# Autodesk Inventor assembly: MACHINEVISE
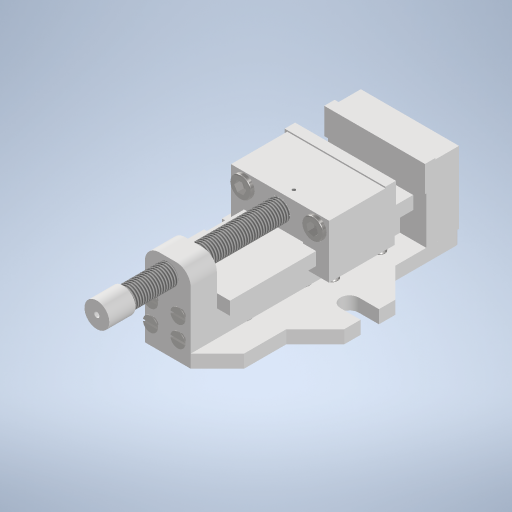
[picture p0: Inventor's stored thumbnail of the model, 512x512]
Saved by Autodesk Inventor 2024 (Build 280153000, 153)
## iProperties
Created: 2023-05-10
Part Number: MACHINEVISE
Document SubType Name: Assembly
Designer: Raj
Author: Raj
## Documents named in this file (16)
- D:\New folder\assembly 2\Assembly\MACHINEVISE.iam
- D:\New folder\assembly 2\Groundplate (1).ipt
- D:\New folder\assembly 2\Spindlesocket.ipt
- D:\New folder\assembly 2\Feste Backe (2).ipt
- D:\New folder\assembly 2\Fuhrung.ipt
- D:\New folder\assembly 2\Lose Backe.ipt
- D:\New folder\assembly 2\Spannbacke(n).ipt
- D:\New folder\assembly 2\Trapezspindle.ipt
- D:\New folder\assembly 2\Druckhulse.ipt
- D:\New folder\assembly 2\Fuhrungschiene(n).ipt
- C:\Users\USER\OneDrive\Documents\Inventor\Content Center Files\R2024\en-US\DIN 963\DIN 963 - M8 x 25.ipt
- C:\Users\USER\OneDrive\Documents\Inventor\Content Center Files\R2024\en-US\DIN 963\DIN 963 - M6 x 25.ipt
- C:\Users\USER\OneDrive\Documents\Inventor\Content Center Files\R2024\en-US\DIN 963\DIN 963 - M6 x 40.ipt
- C:\Users\USER\OneDrive\Documents\Inventor\Content Center Files\R2024\en-US\DIN 963\DIN 963 - M6 x 20.ipt
- C:\Users\USER\OneDrive\Documents\Inventor\Content Center Files\R2024\en-US\DIN 963\DIN 963 - M5 x 16.ipt
- C:\Users\USER\OneDrive\Documents\Inventor\Content Center Files\R2024\en-US\DIN 912\DIN 912 - M10 x 1.5 x 45 x 32.ipt
## Components (32 placed, 15 different names)
1. Groundplate (1):1 — Mate:1, Flush:1, Mate:2, Mate:3, Mate:4, Flush:2, Mate:7, Insert:13, Insert:14, Insert:15, Insert:16, Insert:17, Insert:18
2. Spindlesocket:1 — Mate:1, Flush:1, Mate:2, Mate:5, Mate:10, Insert:7, Insert:8, Insert:9, Insert:10
3. Fuhrung:1 — Mate:3, Mate:4, Mate:5, Mate:6, Mate:9
4. Feste Backe (2):1 — Mate:6, Flush:2, Mate:7, Mate:11, Mate:12, Mate:13, Insert:2, Insert:3, Insert:4, Insert:5, Insert:6
5. Lose Backe:1 — Mate:9, Mate:10, Insert:1, Mate:14, Mate:15, Mate:16, Mate:17, Mate:18, Mate:19, Mate:20, Mate:21, Mate:22, Mate:23, Mate:24, Insert:11, Insert:12
6. Trapezspindle:1 — Insert:1
7. Spannbacke(n):1 — Mate:11, Mate:12, Mate:13
8. Spannbacke(n):2 — Mate:14, Mate:15, Mate:16
9. Druckhulse:1 — Mate:17, Mate:18
10. Fuhrungschiene(n):1 — Mate:19, Mate:20, Mate:21, Insert:19, Insert:20
11. Fuhrungschiene(n):2 — Mate:22, Mate:23, Mate:24, Insert:21, Insert:22
12. DIN 963 - replaced by DIN EN ISO 2009 M8 x 25:1 — Insert:2
13. DIN 963 - replaced by DIN EN ISO 2009 M8 x 25:2 — Insert:3
14. DIN 963 - replaced by DIN EN ISO 2009 M8 x 25:3 — Insert:4
15. DIN 963 - replaced by DIN EN ISO 2009 M6 x 25:1 — Insert:5
16. DIN 963 - replaced by DIN EN ISO 2009 M6 x 25:2 — Insert:6
17. DIN 963 - replaced by DIN EN ISO 2009 M6 x 40:1 — Insert:7
18. DIN 963 - replaced by DIN EN ISO 2009 M6 x 40:2 — Insert:8
19. DIN 963 - replaced by DIN EN ISO 2009 M6 x 40:3 — Insert:10
20. DIN 963 - replaced by DIN EN ISO 2009 M6 x 40:4 — Insert:9
21. DIN 912 - replaced by DIN EN ISO 4762 M10 x 45:1 — Insert:11
22. DIN 912 - replaced by DIN EN ISO 4762 M10 x 45:2 — Insert:12
23. DIN 963 - replaced by DIN EN ISO 2009 M6 x 20:1 — Insert:13
24. DIN 963 - replaced by DIN EN ISO 2009 M6 x 20:2 — Insert:15
25. DIN 963 - replaced by DIN EN ISO 2009 M6 x 20:3 — Insert:17
26. DIN 963 - replaced by DIN EN ISO 2009 M6 x 20:4 — Insert:18
27. DIN 963 - replaced by DIN EN ISO 2009 M6 x 20:5 — Insert:16
28. DIN 963 - replaced by DIN EN ISO 2009 M6 x 20:6 — Insert:14
29. DIN 963 - replaced by DIN EN ISO 2009 M5 x 16:1 — Insert:19
30. DIN 963 - replaced by DIN EN ISO 2009 M5 x 16:2 — Insert:20
31. DIN 963 - replaced by DIN EN ISO 2009 M5 x 16:3 — Insert:21
32. DIN 963 - replaced by DIN EN ISO 2009 M5 x 16:4 — Insert:22
## Relationships (47: Mate 23, Insert 22, Flush 2)
- Mate:1: Groundplate (1):1 ↔ Spindlesocket:1
- Flush:1: Groundplate (1):1 ↔ Spindlesocket:1
- Mate:2: Groundplate (1):1 ↔ Spindlesocket:1
- Mate:3: Groundplate (1):1 ↔ Fuhrung:1
- Mate:4: Groundplate (1):1 ↔ Fuhrung:1
- Mate:5: Spindlesocket:1 ↔ Fuhrung:1
- Mate:6: Fuhrung:1 ↔ Feste Backe (2):1
- Flush:2: Groundplate (1):1 ↔ Feste Backe (2):1
- Mate:7: Groundplate (1):1 ↔ Feste Backe (2):1
- Mate:9: Fuhrung:1 ↔ Lose Backe:1
- Mate:10: Spindlesocket:1 ↔ Lose Backe:1
- Insert:1: Lose Backe:1 ↔ Trapezspindle:1
- Mate:11: Feste Backe (2):1 ↔ Spannbacke(n):1
- Mate:12: Feste Backe (2):1 ↔ Spannbacke(n):1
- Mate:13: Feste Backe (2):1 ↔ Spannbacke(n):1
- Mate:14: Lose Backe:1 ↔ Spannbacke(n):2
- Mate:15: Lose Backe:1 ↔ Spannbacke(n):2
- Mate:16: Lose Backe:1 ↔ Spannbacke(n):2
- Mate:17: Lose Backe:1 ↔ Druckhulse:1
- Mate:18: Lose Backe:1 ↔ Druckhulse:1
- Mate:19: Lose Backe:1 ↔ Fuhrungschiene(n):1
- Mate:20: Lose Backe:1 ↔ Fuhrungschiene(n):1
- Mate:21: Lose Backe:1 ↔ Fuhrungschiene(n):1
- Mate:22: Lose Backe:1 ↔ Fuhrungschiene(n):2
- Mate:23: Lose Backe:1 ↔ Fuhrungschiene(n):2
- Mate:24: Lose Backe:1 ↔ Fuhrungschiene(n):2
- Insert:2: Feste Backe (2):1 ↔ DIN 963 - replaced by DIN EN ISO 2009 M8 x 25:1
- Insert:3: Feste Backe (2):1 ↔ DIN 963 - replaced by DIN EN ISO 2009 M8 x 25:2
- Insert:4: Feste Backe (2):1 ↔ DIN 963 - replaced by DIN EN ISO 2009 M8 x 25:3
- Insert:5: Feste Backe (2):1 ↔ DIN 963 - replaced by DIN EN ISO 2009 M6 x 25:1
- Insert:6: Feste Backe (2):1 ↔ DIN 963 - replaced by DIN EN ISO 2009 M6 x 25:2
- Insert:7: Spindlesocket:1 ↔ DIN 963 - replaced by DIN EN ISO 2009 M6 x 40:1
- Insert:8: Spindlesocket:1 ↔ DIN 963 - replaced by DIN EN ISO 2009 M6 x 40:2
- Insert:9: Spindlesocket:1 ↔ DIN 963 - replaced by DIN EN ISO 2009 M6 x 40:4
- Insert:10: Spindlesocket:1 ↔ DIN 963 - replaced by DIN EN ISO 2009 M6 x 40:3
- Insert:11: Lose Backe:1 ↔ DIN 912 - replaced by DIN EN ISO 4762 M10 x 45:1
- Insert:12: Lose Backe:1 ↔ DIN 912 - replaced by DIN EN ISO 4762 M10 x 45:2
- Insert:13: Groundplate (1):1 ↔ DIN 963 - replaced by DIN EN ISO 2009 M6 x 20:1
- Insert:14: Groundplate (1):1 ↔ DIN 963 - replaced by DIN EN ISO 2009 M6 x 20:6
- Insert:15: Groundplate (1):1 ↔ DIN 963 - replaced by DIN EN ISO 2009 M6 x 20:2
- Insert:16: Groundplate (1):1 ↔ DIN 963 - replaced by DIN EN ISO 2009 M6 x 20:5
- Insert:17: Groundplate (1):1 ↔ DIN 963 - replaced by DIN EN ISO 2009 M6 x 20:3
- Insert:18: Groundplate (1):1 ↔ DIN 963 - replaced by DIN EN ISO 2009 M6 x 20:4
- Insert:19: Fuhrungschiene(n):1 ↔ DIN 963 - replaced by DIN EN ISO 2009 M5 x 16:1
- Insert:20: Fuhrungschiene(n):1 ↔ DIN 963 - replaced by DIN EN ISO 2009 M5 x 16:2
- Insert:21: Fuhrungschiene(n):2 ↔ DIN 963 - replaced by DIN EN ISO 2009 M5 x 16:3
- Insert:22: Fuhrungschiene(n):2 ↔ DIN 963 - replaced by DIN EN ISO 2009 M5 x 16:4
